# Autodesk Inventor assembly: 1310162 DHRS-25-A---(0)
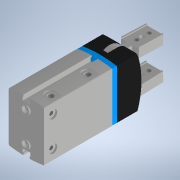
[picture p0: Inventor's stored thumbnail of the model, 180x180]
Saved by Autodesk Inventor 2021 (Build 250183000, 183)
## iProperties
Category: PARTsolutions
Company: FESTO
Created: 2025-06-13
Part Number: 1310162 DHRS-25-A---(0)
Catalog Web Link: www.cadenas.de
Description: DHRS-Radial gripper
Vendor: FESTO
Document SubType Name: Assembly
Designer: psAdmin
Manufacturer: FESTO
Mass: 270 g
Surface Area: 232.155 cm^2
Volume: 103.283 cm^3
Density: 2.61417 g/cm^3
Title: 1310162 DHRS-25-A
Author: Cadenas PARTsolutions
Comments: Radial gripper
PSOL_IDENT_0: {ATYP=ASSISTANT},{DATA=script=$CADENAS_DATA/23d-libs/festo/webfesto.vbb&M_FAMILY=DHRS&M_GROUP=01&M_P
PSOL_IDENT_1: ARTNO=1310162&IDCODE1=DHRS-25-A&IDCODE2=&customer_number_cns=&MATES=1&LOD=HI&LOCKERP=0&SINGLEPART=1}
NB: 1310162 DHRS-25-A---(0)
NN: DHRS
NT: Radial gripper
NBSYN: $TNR. $TYP.---($ROT.)
LINA: 1310162 DHRS-25-A
CATALOG: Festo
TNR: 1310162
TYP: DHRS-25-A
ROT: 0
B1: 29.5
B2: 0
B3: 8.75
B4: 15
B5: 13
D1: 3
D2: 3.3
D3: 7
D4: 9
D5: M4
D6: M4
D7: 7
D8: 5.3
EE: M5
H1: 107.2
H2: 84
H3: 57
H4: 89.45
H5: 21.2
H6: 24.95
H7: 10.25
H8: 5.25
H9: 10.5
H10: 7.5
H11: 11.8
H12: 31
H13: 9
L1: 44
L2: 25
L3: 22.2
L4: 23.2
L5: 6
L6: 1
L7: 8
T1: 1.6
T2: 6.4
T3: 4.5
T4: 21
T5: 1.4
W1: 90
W2: 2
CNSMASSEXACT: 0.27
GTIN: 4052568229597
SUPPLIER: FESTO
ARTICLENO: 1310162 DHRS-25-A---(0)
BOMINFO: 1310162 DHRS-25-A
CREATOR: CADENAS GmbH
## Documents named in this file (4)
- e:\temp\worker_COMMON_10\temp\tmp_5004_0_hi4bt\format_0\1310162 DHRS-25-A---(0).iam
- e:\temp\worker_COMMON_10\temp\tmp_5004_0_hi4bt\format_0\1310162 DHRS-25-A---(Geh).ipt
- e:\temp\worker_COMMON_10\temp\tmp_5004_0_hi4bt\format_0\1310162 DHRS-25-A---(Griff).ipt
- e:\temp\worker_COMMON_10\temp\tmp_5004_0_hi4bt\format_0\8146544 ZBH-7-B.ipt
## Components (5 placed, 3 different names)
1. 1310162 DHRS-25-A---(Geh):1 — TO_JAW_L_XY@1 <-> GRIFF_XY@2, TO_JAW_L_Z@1 <-> GRIFF_Z@2, TO_JAW_L_YZ@1 <-> GRIFF_YZ@2, TO_JAW_R_XY@1 <-> GRIFF_XY@3, TO_JAW_R_Z@1 <-> GRIFF_Z@3, TO_JAW_R_YZ@1 <-> GRIFF_YZ@3, TO_ZBH_1_Z@1 <-> insert_Z@4, TO_ZBH_1_YZ@1 <-> insert_YZ@4, TO_ZBH_2_Z@1 <-> insert_Z@5, TO_ZBH_2_YZ@1 <-> insert_YZ@5
2. 1310162 DHRS-25-A---(Griff):1 — TO_JAW_L_XY@1 <-> GRIFF_XY@2, TO_JAW_L_Z@1 <-> GRIFF_Z@2, TO_JAW_L_YZ@1 <-> GRIFF_YZ@2
3. 1310162 DHRS-25-A---(Griff):2 — TO_JAW_R_XY@1 <-> GRIFF_XY@3, TO_JAW_R_Z@1 <-> GRIFF_Z@3, TO_JAW_R_YZ@1 <-> GRIFF_YZ@3
4. 8146544 ZBH-7-B:1 — TO_ZBH_1_Z@1 <-> insert_Z@4, TO_ZBH_1_YZ@1 <-> insert_YZ@4
5. 8146544 ZBH-7-B:2 — TO_ZBH_2_Z@1 <-> insert_Z@5, TO_ZBH_2_YZ@1 <-> insert_YZ@5
## Relationships (10: Mate 5, Angle 4, Flush 1)
- TO_JAW_L_XY@1 <-> GRIFF_XY@2 [Flush]: 1310162 DHRS-25-A---(Geh):1 ↔ 1310162 DHRS-25-A---(Griff):1
- TO_JAW_L_Z@1 <-> GRIFF_Z@2 [Mate]: 1310162 DHRS-25-A---(Geh):1 ↔ 1310162 DHRS-25-A---(Griff):1
- TO_JAW_L_YZ@1 <-> GRIFF_YZ@2 [Angle] (-2 deg): 1310162 DHRS-25-A---(Geh):1 ↔ 1310162 DHRS-25-A---(Griff):1
- TO_JAW_R_XY@1 <-> GRIFF_XY@3 [Mate]: 1310162 DHRS-25-A---(Geh):1 ↔ 1310162 DHRS-25-A---(Griff):2
- TO_JAW_R_Z@1 <-> GRIFF_Z@3 [Mate]: 1310162 DHRS-25-A---(Geh):1 ↔ 1310162 DHRS-25-A---(Griff):2
- TO_JAW_R_YZ@1 <-> GRIFF_YZ@3 [Angle] (182 deg): 1310162 DHRS-25-A---(Geh):1 ↔ 1310162 DHRS-25-A---(Griff):2
- TO_ZBH_1_Z@1 <-> insert_Z@4 [Mate]: 1310162 DHRS-25-A---(Geh):1 ↔ 8146544 ZBH-7-B:1
- TO_ZBH_1_YZ@1 <-> insert_YZ@4 [Angle] (0 deg): 1310162 DHRS-25-A---(Geh):1 ↔ 8146544 ZBH-7-B:1
- TO_ZBH_2_Z@1 <-> insert_Z@5 [Mate]: 1310162 DHRS-25-A---(Geh):1 ↔ 8146544 ZBH-7-B:2
- TO_ZBH_2_YZ@1 <-> insert_YZ@5 [Angle] (0 deg): 1310162 DHRS-25-A---(Geh):1 ↔ 8146544 ZBH-7-B:2
